# Autodesk Inventor assembly: ŚRUBA + PODKŁADKI + NAKRĘTKA
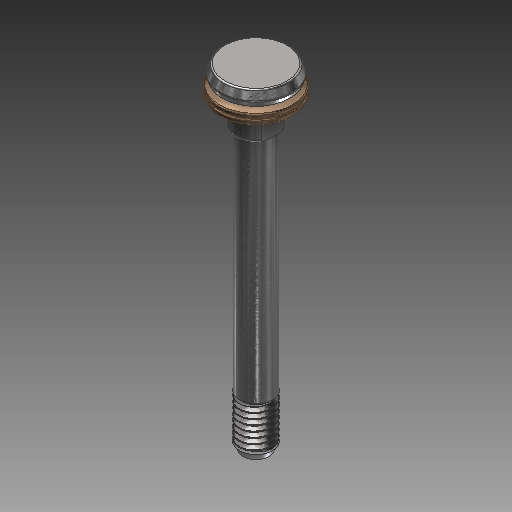
[picture p0: Inventor's stored thumbnail of the model, 512x512]
Saved by Autodesk Inventor 2017 SP1 (Build 210196100, 196)
## iProperties
Created: 2021-02-09
Part Number: ŚRUBA + PODKŁADKI + NAKRĘTKA
Document SubType Name: Assembly
Designer: Napoleon
Author: Napoleon
## Documents named in this file (3)
- D:\PRYWATNE\PROJEKTY\POKÓJ\URZĄDZENIA PERYFERYJNE\DELL 1909Wf\ŚRUBA + PODKŁADKI + NAKRĘTKA.iam
- D:\PRYWATNE\PROJEKTY\POKÓJ\URZĄDZENIA PERYFERYJNE\DELL 1909Wf\ŚRUBA KOSZYKA.ipt
- D:\PRYWATNE\PROJEKTY\POKÓJ\URZĄDZENIA PERYFERYJNE\DELL 1909Wf\PODKŁADKA M6x11.ipt
## Components (3 placed, 2 different names)
1. ŚRUBA KOSZYKA:1 — Zestawiający:3
2. PODKŁADKA M6x11:1 — Zestawiający:3, Zestawiający:4
3. PODKŁADKA M6x11:2 — Zestawiający:4
## Relationships (2: Mate 2)
- Zestawiający:3 [Mate]: ŚRUBA KOSZYKA:1 ↔ PODKŁADKA M6x11:1
- Zestawiający:4 [Mate]: PODKŁADKA M6x11:1 ↔ PODKŁADKA M6x11:2
